# Autodesk Inventor assembly: MGN12H_With_Rail
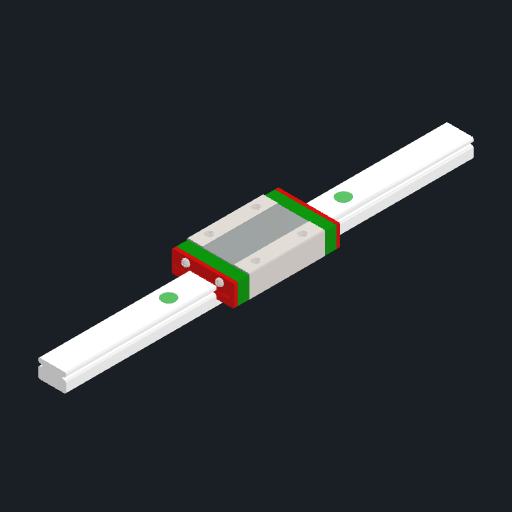
[picture p0: Inventor's stored thumbnail of the model, 512x512]
Saved by Autodesk Inventor 2026.2 (Build 302298000, 298)
## iProperties
Created: 2026-02-12
Part Number: MGN12H_With_Rail
Description: STEP AP214
Document SubType Name: Assembly
Designer: AdminForWorker
Title: MGN12H_With_Rail y axis v1
Author: AdminForWorker
## Documents named in this file (5)
- C:\Users\Alvin\OneDrive\Documents\Inventor\NCKU_Automation_Incubator_Microscope\MGN12H_With_Rail y axis\MGN12H_With_Rail y axis.iam
- C:\Users\Alvin\OneDrive\Documents\Inventor\NCKU_Automation_Incubator_Microscope\MGN12H_With_Rail y axis\MGNR12R100HM.ipt
- C:\Users\Alvin\OneDrive\Documents\Inventor\NCKU_Automation_Incubator_Microscope\MGN12H_With_Rail y axis\MGN12H.iam
- C:\Users\Alvin\OneDrive\Documents\Inventor\NCKU_Automation_Incubator_Microscope\MGN12H_With_Rail y axis\Screw_DIN_912_M3x8F_A2.ipt
- C:\Users\Alvin\OneDrive\Documents\Inventor\NCKU_Automation_Incubator_Microscope\MGN12H_With_Rail y axis\MGN12R_CoverCap.ipt
## Components (10 placed, 4 different names)
1. MGNR12R100HM:1 — Slider:1, Mate:9, Mate:10, Mate:11, Mate:12, Flush:1, Flush:2, Flush:3, Flush:4
2. MGN12H:1 [sub-assembly] — Slider:1
3. Screw_DIN_912_M3x8F_A2:1 — Mate:1, Mate:2, Mate:12
4. MGN12R_CoverCap:1 — Mate:1, Mate:2, Flush:4
5. Screw_DIN_912_M3x8F_A2:2 — Mate:3, Mate:6, Mate:11
6. Screw_DIN_912_M3x8F_A2:3 — Mate:4, Mate:7, Mate:9
7. Screw_DIN_912_M3x8F_A2:4 — Mate:5, Mate:8, Mate:10
8. MGN12R_CoverCap:2 — Mate:3, Mate:6, Flush:1
9. MGN12R_CoverCap:3 — Mate:4, Mate:7, Flush:2
10. MGN12R_CoverCap:4 — Mate:5, Mate:8, Flush:3
## Relationships (17: Mate 12, Flush 4, TranslationJoint 1)
- Slider:1 [TranslationJoint]: MGNR12R100HM:1 ↔ MGN12H:1
- Mate:1: Screw_DIN_912_M3x8F_A2:1 ↔ MGN12R_CoverCap:1
- Mate:2: Screw_DIN_912_M3x8F_A2:1 ↔ MGN12R_CoverCap:1
- Mate:3: Screw_DIN_912_M3x8F_A2:2 ↔ MGN12R_CoverCap:2
- Mate:4: Screw_DIN_912_M3x8F_A2:3 ↔ MGN12R_CoverCap:3
- Mate:5: Screw_DIN_912_M3x8F_A2:4 ↔ MGN12R_CoverCap:4
- Mate:6: Screw_DIN_912_M3x8F_A2:2 ↔ MGN12R_CoverCap:2
- Mate:7: Screw_DIN_912_M3x8F_A2:3 ↔ MGN12R_CoverCap:3
- Mate:8: Screw_DIN_912_M3x8F_A2:4 ↔ MGN12R_CoverCap:4
- Mate:9: MGNR12R100HM:1 ↔ Screw_DIN_912_M3x8F_A2:3
- Mate:10: MGNR12R100HM:1 ↔ Screw_DIN_912_M3x8F_A2:4
- Mate:11: MGNR12R100HM:1 ↔ Screw_DIN_912_M3x8F_A2:2
- Mate:12: MGNR12R100HM:1 ↔ Screw_DIN_912_M3x8F_A2:1
- Flush:1: MGNR12R100HM:1 ↔ MGN12R_CoverCap:2
- Flush:2: MGNR12R100HM:1 ↔ MGN12R_CoverCap:3
- Flush:3: MGNR12R100HM:1 ↔ MGN12R_CoverCap:4
- Flush:4: MGNR12R100HM:1 ↔ MGN12R_CoverCap:1
